# Autodesk Inventor assembly: hydraulic_jack_system
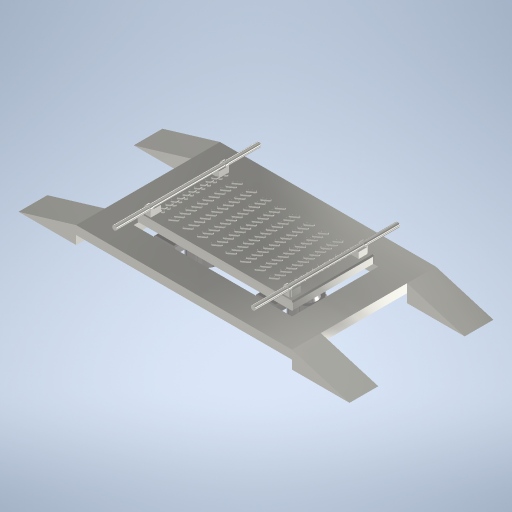
[picture p0: Inventor's stored thumbnail of the model, 512x512]
Saved by Autodesk Inventor 2023 (Build 270158000, 158)
## iProperties
Created: 2023-11-22
Part Number: hydraulic_jack_system
Document SubType Name: Assembly
Designer: Beatrice
Author: Beatrice
## Documents named in this file (4)
- E:\WORKSPACE_2\wheel_changing_assignment\hydraulic_jack_system.iam
- E:\WORKSPACE_2\wheel_changing_assignment\Base_plartform.ipt
- E:\WORKSPACE_2\wheel_changing_assignment\hydraulic_cylinder.iam
- E:\WORKSPACE_2\wheel_changing_assignment\middle_base_Platform.ipt
## Components (4 placed, 3 different names)
1. Base_plartform:1 — Flush:3, Flush:4, Flush:5
2. hydraulic_cylinder:1 [sub-assembly] — Flush:1, Flush:2, Mate:1, Flush:5
3. hydraulic_cylinder:2 [sub-assembly] — Flush:1, Flush:2, Mate:2, Mate:3
4. middle_base_Platform:1 — Mate:1, Mate:2, Mate:3, Flush:3, Flush:4
## Relationships (8: Flush 5, Mate 3)
- Flush:1: hydraulic_cylinder:1 ↔ hydraulic_cylinder:2
- Flush:2: hydraulic_cylinder:1 ↔ hydraulic_cylinder:2
- Mate:1: hydraulic_cylinder:1 ↔ middle_base_Platform:1
- Mate:2: hydraulic_cylinder:2 ↔ middle_base_Platform:1
- Mate:3: hydraulic_cylinder:2 ↔ middle_base_Platform:1
- Flush:3: Base_plartform:1 ↔ middle_base_Platform:1
- Flush:4: Base_plartform:1 ↔ middle_base_Platform:1
- Flush:5 (30 mm): Base_plartform:1 ↔ hydraulic_cylinder:1
